# Autodesk Inventor assembly: platform_0606_fig2_ratio12
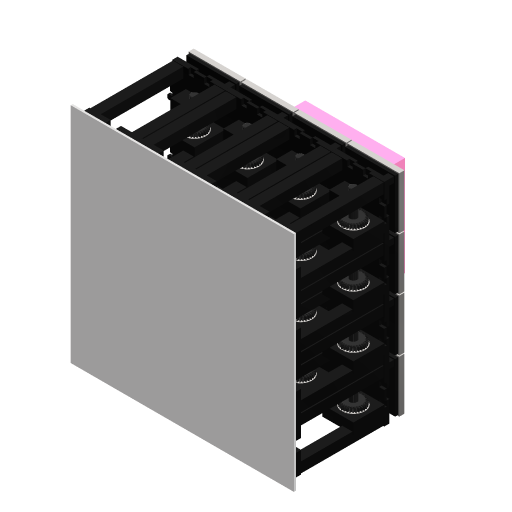
[picture p0: Inventor's stored thumbnail of the model, 512x512]
Saved by Autodesk Inventor 2024 (Build 280153000, 153)
## iProperties
Created: 2024-06-06
Part Number: platform_0606_fig2_ratio12
Document SubType Name: Assembly
Designer: admin
Author: admin
## Documents named in this file (9)
- C:\Users\admin\OneDrive\文件\碩士研究\prototype\plane_unit_0606\platform_0606_fig2_ratio18.iam
- C:\Users\admin\OneDrive\文件\碩士研究\prototype\plane_unit_0606\one_way_bearing.ipt
- C:\Users\admin\OneDrive\文件\碩士研究\prototype\plane_unit_0606\printer_base_plane.ipt
- C:\Users\admin\OneDrive\文件\碩士研究\prototype\plane_unit_0606\rod_1221.ipt
- C:\Users\admin\OneDrive\文件\碩士研究\prototype\plane_unit_0606\iron_plate.ipt
- C:\Users\admin\OneDrive\文件\碩士研究\prototype\plane_unit_0606\plane_unit_1121.ipt
- C:\Users\admin\OneDrive\文件\碩士研究\prototype\plane_unit_0606\gear_pin_1222_.ipt
- C:\Users\admin\OneDrive\文件\碩士研究\prototype\plane_unit_0606\bridge_rect_final_12.ipt
- C:\Users\admin\OneDrive\文件\碩士研究\prototype\plane_unit_0606\trimmed_block_12.ipt
## Components (83 placed, 8 different names)
1. printer_base_plane:1 — 貼合:1, 齊平:1, 齊平:2, 齊平:4, 齊平:5, 25, 貼合:12
2. bridge_rect_final_12:1 — 齊平:5, 25, 貼合:12, 貼合:13, 齊平:7, 貼合:14
3. trimmed_block_12:1 — 貼合:13, 齊平:7, 貼合:14
4. iron_plate:1 — 貼合:9, 貼合:10, 貼合:11, 齊平:4
5. rod_1221:1 — 貼合:7, 貼合:8, 貼合:9, 貼合:10, 貼合:11
6. gear_pin_1222_:1 — 貼合:3, 貼合:4
7. plane_unit_1121:1 — 貼合:1, 齊平:1, 齊平:2, 貼合:2, 齊平:3, 貼合:7, 貼合:8
8. one_way_bearing:1 — 貼合:2, 齊平:3, 貼合:3, 貼合:4
9. iron_plate:2
10. rod_1221:2
11. gear_pin_1222_:2
12. plane_unit_1121:2
13. one_way_bearing:2
14. iron_plate:3
15. rod_1221:3
16. gear_pin_1222_:3
17. plane_unit_1121:3
18. one_way_bearing:3
19. iron_plate:4
20. rod_1221:4
21. gear_pin_1222_:4
22. plane_unit_1121:4
23. one_way_bearing:4
24. iron_plate:5
25. rod_1221:5
26. gear_pin_1222_:5
27. plane_unit_1121:5
28. one_way_bearing:5
29. iron_plate:6
30. rod_1221:6
31. gear_pin_1222_:6
32. plane_unit_1121:6
33. one_way_bearing:6
34. iron_plate:7
35. rod_1221:7
36. gear_pin_1222_:7
37. plane_unit_1121:7
38. one_way_bearing:7
39. iron_plate:8
40. rod_1221:8
41. gear_pin_1222_:8
42. plane_unit_1121:8
43. one_way_bearing:8
44. iron_plate:9
45. rod_1221:9
46. gear_pin_1222_:9
47. plane_unit_1121:9
48. one_way_bearing:9
49. iron_plate:10
50. rod_1221:10
51. gear_pin_1222_:10
52. plane_unit_1121:10
53. one_way_bearing:10
54. iron_plate:11
55. rod_1221:11
56. gear_pin_1222_:11
57. plane_unit_1121:11
58. one_way_bearing:11
59. iron_plate:12
60. rod_1221:12
61. gear_pin_1222_:12
62. plane_unit_1121:12
63. one_way_bearing:12
64. iron_plate:13
65. rod_1221:13
66. gear_pin_1222_:13
67. plane_unit_1121:13
68. one_way_bearing:13
69. iron_plate:14
70. rod_1221:14
71. gear_pin_1222_:14
72. plane_unit_1121:14
73. one_way_bearing:14
74. iron_plate:15
75. rod_1221:15
76. gear_pin_1222_:15
77. plane_unit_1121:15
78. one_way_bearing:15
79. iron_plate:16
80. rod_1221:16
81. gear_pin_1222_:16
82. plane_unit_1121:16
83. one_way_bearing:16
## Component patterns: (16 elements, first: iron_plate:1 + rod_1221:1 + gear_pin_1222_:1 + plane_unit_1121:1 + one_way_bearing:1)
## Relationships (19: Mate 12, Flush 7)
- 貼合:1 [Mate]: printer_base_plane:1 ↔ plane_unit_1121:1
- 齊平:1 [Flush] (5 mm): printer_base_plane:1 ↔ plane_unit_1121:1
- 齊平:2 [Flush] (5 mm): printer_base_plane:1 ↔ plane_unit_1121:1
- 貼合:2 [Mate]: plane_unit_1121:1 ↔ one_way_bearing:1
- 齊平:3 [Flush]: plane_unit_1121:1 ↔ one_way_bearing:1
- 貼合:3 [Mate]: gear_pin_1222_:1 ↔ one_way_bearing:1
- 貼合:4 [Mate]: gear_pin_1222_:1 ↔ one_way_bearing:1
- 貼合:7 [Mate] (0.2 mm): rod_1221:1 ↔ plane_unit_1121:1
- 貼合:8 [Mate] (0.2 mm): rod_1221:1 ↔ plane_unit_1121:1
- 貼合:9 [Mate]: iron_plate:1 ↔ rod_1221:1
- 貼合:10 [Mate]: iron_plate:1 ↔ rod_1221:1
- 貼合:11 [Mate]: iron_plate:1 ↔ rod_1221:1
- 齊平:4 [Flush] (-110 mm): printer_base_plane:1 ↔ iron_plate:1
- 齊平:5 [Flush] (35 mm): printer_base_plane:1 ↔ bridge_rect_final_12:1
- 25 [Flush] (25 mm): printer_base_plane:1 ↔ bridge_rect_final_12:1
- 貼合:12 [Mate] (110 mm): printer_base_plane:1 ↔ bridge_rect_final_12:1
- 貼合:13 [Mate]: bridge_rect_final_12:1 ↔ trimmed_block_12:1
- 齊平:7 [Flush]: bridge_rect_final_12:1 ↔ trimmed_block_12:1
- 貼合:14 [Mate]: bridge_rect_final_12:1 ↔ trimmed_block_12:1
